# Autodesk Inventor assembly: Final Project Assembly
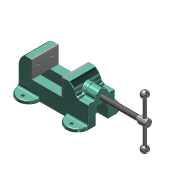
[picture p0: Inventor's stored thumbnail of the model, 180x180]
Saved by Autodesk Inventor 2017 (Build 210142000, 142)
## iProperties
Created: 2016-12-09
Part Number: Final Project Assembly
Document SubType Name: Assembly
Designer: Lince
Author: Lince
## Documents named in this file (13)
- C:\Users\Lince\Documents\Fall 2016\Engr Principles\Final Project - Vise\Final Project Assembly.iam
- C:\Users\Lince\Documents\Fall 2016\Engr Principles\Final Project - Vise\VS-001 (BASE).ipt
- C:\Users\Lince\Documents\Fall 2016\Engr Principles\Final Project - Vise\VS-002 (SLIDING JAW).ipt
- C:\Users\Lince\Documents\Fall 2016\Engr Principles\Final Project - Vise\VS-003 (JAW PLATE).ipt
- C:\Users\Lince\Documents\Fall 2016\Engr Principles\Final Project - Vise\VS-004 (VISE SCREW).ipt
- C:\Users\Lince\Documents\Fall 2016\Engr Principles\Final Project - Vise\VS-005(COLLAR).ipt
- C:\Users\Lince\Documents\Fall 2016\Engr Principles\Final Project - Vise\VS-006 (SPECIAL KEY).ipt
- C:\Users\Lince\Documents\Fall 2016\Engr Principles\Final Project - Vise\VS-007 (HANDLE ROD).ipt
- C:\Users\Lince\Documents\Fall 2016\Engr Principles\Final Project - Vise\VS-008 (HANDLE BALL).ipt
- C:\Users\Lince\Documents\Fall 2016\Engr Principles\Final Project - Vise\VS-009 (SLIDE KEY).ipt
- C:\Users\Lince\Documents\Fall 2016\Engr Principles\Final Project - Vise\VS-010 (SET SCREW).ipt
- C:\Users\Lince\Documents\Fall 2016\Engr Principles\Final Project - Vise\ANSI B18.6.2 - 1_4-20 UNC - 0.75.ipt
- C:\Users\Lince\Documents\Fall 2016\Engr Principles\Final Project - Vise\ANSI B18.8.2 - No. 2_0 x 3_4  0.1423.ipt
## Components (20 placed, 12 different names)
1. VS-001 (BASE):1 — Mate:1, Mate:2, Mate:3, Mate:4, Mate:5, Mate:6
2. VS-002 (SLIDING JAW):1 — Mate:1, Mate:2, Mate:3, Mate:7, Flush:1, Flush:2, Mate:18, Mate:19, Mate:20, Mate:26, Mate:27, Mate:28, Mate:29, Mate:30, Mate:31, Mate:32, Mate:33, Mate:34, Mate:35
3. VS-003 (JAW PLATE):1 — Mate:4, Mate:5, Mate:6, Insert:5, Insert:6
4. VS-003 (JAW PLATE):2 — Mate:7, Flush:1, Flush:2, Insert:3, Insert:4
5. VS-004 (VISE SCREW):1 — Mate:8, Mate:9, Mate:10, Mate:12, Mate:13, Mate:14, Mate:17, Mate:18, Mate:19, Mate:20, Mate:21
6. VS-005(COLLAR):1 — Mate:11, Mate:12
7. VS-006 (SPECIAL KEY):1 — Mate:8, Mate:9, Mate:10, Mate:11, Mate:17
8. VS-007 (HANDLE ROD):1 — Mate:13, Mate:14, Insert:1, Mate:15, Insert:2, Mate:16, Mate:21
9. VS-008 (HANDLE BALL):1 — Insert:1, Mate:15, Insert:7
10. VS-008 (HANDLE BALL):2 — Insert:2, Mate:16, Insert:8
11. VS-009 (SLIDE KEY):1 — Mate:29, Mate:30, Mate:31
12. VS-009 (SLIDE KEY):2 — Mate:26, Mate:27, Mate:28
13. VS-010 (SET SCREW):1 — Mate:32, Mate:33
14. VS-010 (SET SCREW):2 — Mate:34, Mate:35
15. Slotted Flat Countersunk Head Cap Screw - Inch 1/4-20 UNC x 0.75:1 — Insert:3, Mate:36
16. Slotted Flat Countersunk Head Cap Screw - Inch 1/4-20 UNC x 0.75:2 — Insert:4, Mate:36
17. Slotted Flat Countersunk Head Cap Screw - Inch 1/4-20 UNC x 0.75:3 — Insert:5, Mate:37
18. Slotted Flat Countersunk Head Cap Screw - Inch 1/4-20 UNC x 0.75:4 — Insert:6, Mate:37
19. Pin - Taper (Inch) No. 2/0 x 3/4:1 — Insert:7
20. Pin - Taper (Inch) No. 2/0 x 3/4:2 — Insert:8
## Relationships (43: Mate 33, Insert 8, Flush 2)
- Mate:1: VS-001 (BASE):1 ↔ VS-002 (SLIDING JAW):1
- Mate:2: VS-001 (BASE):1 ↔ VS-002 (SLIDING JAW):1
- Mate:3: VS-001 (BASE):1 ↔ VS-002 (SLIDING JAW):1
- Mate:4: VS-001 (BASE):1 ↔ VS-003 (JAW PLATE):1
- Mate:5: VS-001 (BASE):1 ↔ VS-003 (JAW PLATE):1
- Mate:6: VS-001 (BASE):1 ↔ VS-003 (JAW PLATE):1
- Mate:7: VS-002 (SLIDING JAW):1 ↔ VS-003 (JAW PLATE):2
- Flush:1: VS-002 (SLIDING JAW):1 ↔ VS-003 (JAW PLATE):2
- Flush:2: VS-002 (SLIDING JAW):1 ↔ VS-003 (JAW PLATE):2
- Mate:8: VS-004 (VISE SCREW):1 ↔ VS-006 (SPECIAL KEY):1
- Mate:9: VS-004 (VISE SCREW):1 ↔ VS-006 (SPECIAL KEY):1
- Mate:10: VS-004 (VISE SCREW):1 ↔ VS-006 (SPECIAL KEY):1
- Mate:11: VS-005(COLLAR):1 ↔ VS-006 (SPECIAL KEY):1
- Mate:12: VS-004 (VISE SCREW):1 ↔ VS-005(COLLAR):1
- Mate:13: VS-004 (VISE SCREW):1 ↔ VS-007 (HANDLE ROD):1
- Mate:14: VS-004 (VISE SCREW):1 ↔ VS-007 (HANDLE ROD):1
- Insert:1: VS-007 (HANDLE ROD):1 ↔ VS-008 (HANDLE BALL):1
- Mate:15: VS-007 (HANDLE ROD):1 ↔ VS-008 (HANDLE BALL):1
- Insert:2: VS-007 (HANDLE ROD):1 ↔ VS-008 (HANDLE BALL):2
- Mate:16: VS-007 (HANDLE ROD):1 ↔ VS-008 (HANDLE BALL):2
- Mate:17: VS-004 (VISE SCREW):1 ↔ VS-006 (SPECIAL KEY):1
- Mate:18: VS-002 (SLIDING JAW):1 ↔ VS-004 (VISE SCREW):1
- Mate:19: VS-002 (SLIDING JAW):1 ↔ VS-004 (VISE SCREW):1
- Mate:20: VS-002 (SLIDING JAW):1 ↔ VS-004 (VISE SCREW):1
- Mate:21: VS-004 (VISE SCREW):1 ↔ VS-007 (HANDLE ROD):1
- Mate:26: VS-002 (SLIDING JAW):1 ↔ VS-009 (SLIDE KEY):2
- Mate:27: VS-002 (SLIDING JAW):1 ↔ VS-009 (SLIDE KEY):2
- Mate:28: VS-002 (SLIDING JAW):1 ↔ VS-009 (SLIDE KEY):2
- Mate:29: VS-002 (SLIDING JAW):1 ↔ VS-009 (SLIDE KEY):1
- Mate:30: VS-002 (SLIDING JAW):1 ↔ VS-009 (SLIDE KEY):1
- Mate:31: VS-002 (SLIDING JAW):1 ↔ VS-009 (SLIDE KEY):1
- Mate:32: VS-002 (SLIDING JAW):1 ↔ VS-010 (SET SCREW):1
- Mate:33: VS-002 (SLIDING JAW):1 ↔ VS-010 (SET SCREW):1
- Mate:34: VS-002 (SLIDING JAW):1 ↔ VS-010 (SET SCREW):2
- Mate:35: VS-002 (SLIDING JAW):1 ↔ VS-010 (SET SCREW):2
- Insert:3: VS-003 (JAW PLATE):2 ↔ Slotted Flat Countersunk Head Cap Screw - Inch 1/4-20 UNC x 0.75:1
- Insert:4: VS-003 (JAW PLATE):2 ↔ Slotted Flat Countersunk Head Cap Screw - Inch 1/4-20 UNC x 0.75:2
- Insert:5: VS-003 (JAW PLATE):1 ↔ Slotted Flat Countersunk Head Cap Screw - Inch 1/4-20 UNC x 0.75:3
- Insert:6: VS-003 (JAW PLATE):1 ↔ Slotted Flat Countersunk Head Cap Screw - Inch 1/4-20 UNC x 0.75:4
- Mate:36: Slotted Flat Countersunk Head Cap Screw - Inch 1/4-20 UNC x 0.75:1 ↔ Slotted Flat Countersunk Head Cap Screw - Inch 1/4-20 UNC x 0.75:2
- Mate:37: Slotted Flat Countersunk Head Cap Screw - Inch 1/4-20 UNC x 0.75:3 ↔ Slotted Flat Countersunk Head Cap Screw - Inch 1/4-20 UNC x 0.75:4
- Insert:7: VS-008 (HANDLE BALL):1 ↔ Pin - Taper (Inch) No. 2/0 x 3/4:1
- Insert:8: VS-008 (HANDLE BALL):2 ↔ Pin - Taper (Inch) No. 2/0 x 3/4:2
